# Autodesk Inventor assembly: B3M-SC-1170-A_with_ClampHorn_AND_FreeHorn
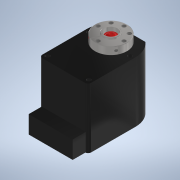
[picture p0: Inventor's stored thumbnail of the model, 180x180]
Saved by Autodesk Inventor 2020 (Build 240168000, 168)
## iProperties
Created: 2022-03-18
Part Number: B3M-SC-1170-A_with_ClampHorn_AND_FreeHorn
Document SubType Name: Assembly
Designer: MasatoKubotera
Author: MasatoKubotera
## Documents named in this file (4)
- C:\Users\MasatoKubotera\Documents\Inventor\SUSTAINA-OP\ReadyMade\KONDO\B3M-SC-1170-A_with_ClampHorn_AND_FreeHorn.iam
- C:\Users\MasatoKubotera\Documents\Inventor\SUSTAINA-OP\ReadyMade\KONDO\B3M-SC-1170-A_with_ClampHorn.iam
- C:\Users\MasatoKubotera\Documents\Inventor\SUSTAINA-OP\ReadyMade\KONDO\FreeHorn.ipt
- C:\Users\MasatoKubotera\Documents\Inventor\SUSTAINA-OP\ReadyMade\KONDO\FreeHorn_Screw.ipt
## Components (3 placed, 3 different names)
1. B3M-SC-1170-A_with_ClampHorn:1 [sub-assembly] — 挿入:1, 挿入:2, フラッシュ:1, フラッシュ:2, フラッシュ:4
2. FreeHorn_:1 — 挿入:1
3. FreeHorn_Screw:1 — 挿入:2
## Relationships (6: Flush 4, Insert 2)
- 挿入:1 [Insert]: B3M-SC-1170-A_with_ClampHorn:1 ↔ FreeHorn_:1
- 挿入:2 [Insert]: B3M-SC-1170-A_with_ClampHorn:1 ↔ FreeHorn_Screw:1
- フラッシュ:1 [Flush]: B3M-SC-1170-A_with_ClampHorn:1
- フラッシュ:2 [Flush]: B3M-SC-1170-A_with_ClampHorn:1
- フラッシュ:3 [Flush]
- フラッシュ:4 [Flush] (-19.75 mm): B3M-SC-1170-A_with_ClampHorn:1
